# Autodesk Inventor assembly: Remote
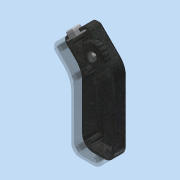
[picture p0: Inventor's stored thumbnail of the model, 180x180]
Saved by Autodesk Inventor 2015 (Build 190159000, 159)
## iProperties
Created: 2015-11-12
Part Number: Remote
Document SubType Name: Assembly
Designer: Raphael
Author: Raphael
## Documents named in this file (5)
- \\psf\Home\Documents\electric-skateboard\Remote\CAD\Remote.iam
- \\psf\Home\Documents\electric-skateboard\Remote\CAD\CaseRight.iam
- \\psf\Home\Documents\electric-skateboard\Remote\CAD\Wheel.iam
- \\psf\Home\Documents\electric-skateboard\Remote\CAD\CaseLeft.iam
- \\psf\Home\Documents\electric-skateboard\Remote\CAD\Button.ipt
## Components (4 placed, 4 different names)
1. CaseRight:1 [sub-assembly] — Mate:1, Mate:2, Mate:3, Mate:4, Mate:5, Mate:6, Mate:7, Mate:8
2. Wheel:1 [sub-assembly] — Mate:1, Mate:2
3. CaseLeft:1 [sub-assembly] — Mate:3, Mate:4, Mate:5
4. Button:1 — Mate:6, Mate:7, Mate:8
## Relationships (8: Mate 8)
- Mate:1: CaseRight:1 ↔ Wheel:1
- Mate:2 (0.7937 mm): CaseRight:1 ↔ Wheel:1
- Mate:3: CaseRight:1 ↔ CaseLeft:1
- Mate:4: CaseRight:1 ↔ CaseLeft:1
- Mate:5: CaseRight:1 ↔ CaseLeft:1
- Mate:6 (0.0254 mm): CaseRight:1 ↔ Button:1
- Mate:7 (0.0254 mm): CaseRight:1 ↔ Button:1
- Mate:8: CaseRight:1 ↔ Button:1
